# Autodesk Inventor assembly: Housing_Assembly_V4
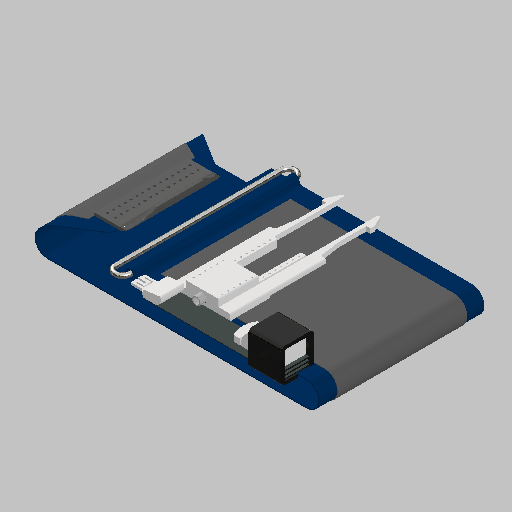
[picture p0: Inventor's stored thumbnail of the model, 512x512]
Saved by Autodesk Inventor 2026.2 (Build 302298000, 298)
## iProperties
Created: 2026-03-15
Part Number: Housing_Assembly_V4
Document SubType Name: Assembly
Designer: vckot
Author: vckot
## Documents named in this file (24)
- C:\Users\vckot\OneDrive\Documents\Vaibhav\capstone\CAD_files\Version_6\Housing_Assembly_V6.iam
- C:\Users\vckot\OneDrive\Documents\Vaibhav\capstone\CAD_files\Version_6\PCB_Housing_01_V4.ipt
- C:\Users\vckot\OneDrive\Documents\Vaibhav\capstone\CAD_files\Version_6\Battery_Small.ipt
- C:\Users\vckot\OneDrive\Documents\Vaibhav\capstone\CAD_files\Version_6\Adafruit_1528_4699_ND.ipt
- C:\Users\vckot\OneDrive\Documents\Vaibhav\capstone\CAD_files\Version_6\Adafruit_1528-4663-ND.ipt
- C:\Users\vckot\OneDrive\Documents\Vaibhav\capstone\CAD_files\Version_6\Adafruit_4662.ipt
- C:\Users\vckot\OneDrive\Documents\Vaibhav\capstone\CAD_files\Version_6\Snap_Switch_Assembly.iam
- C:\Users\vckot\OneDrive\Documents\Vaibhav\capstone\CAD_files\Version_6\PCB_Housing_02_V4.ipt
- C:\Users\vckot\OneDrive\Documents\Vaibhav\capstone\CAD_files\Version_6\PCB_Housing_03_V4.ipt
- C:\Users\vckot\OneDrive\Documents\Vaibhav\capstone\CAD_files\Version_6\PCB_Housing_04_V4.ipt
- C:\Users\vckot\OneDrive\Documents\Vaibhav\capstone\CAD_files\Version_6\TourniquetPCBV1_Updated.iam
- C:\Users\vckot\OneDrive\Documents\Vaibhav\capstone\CAD_files\Version_6\PCB_Housing_05_V4.ipt
- C:\Users\vckot\OneDrive\Documents\Vaibhav\capstone\CAD_files\Version_6\7_Seg_Display_TM1637.ipt
- C:\Users\vckot\OneDrive\Documents\Vaibhav\capstone\CAD_files\Version_6\PCB_Housing_07_V4.ipt
- C:\Users\vckot\OneDrive\Documents\Vaibhav\capstone\CAD_files\Version_6\PCB_Housing_06_V4.ipt
- C:\Users\vckot\OneDrive\Documents\Vaibhav\capstone\CAD_files\Version_6\Tourniquet_Rail_01_V4.ipt
- C:\Users\vckot\OneDrive\Documents\Vaibhav\capstone\CAD_files\Version_6\PCB_Housing_08_V4.ipt
- C:\Users\vckot\OneDrive\Documents\Vaibhav\capstone\CAD_files\Version_6\Tubing_Male_Connector.ipt
- C:\Users\vckot\OneDrive\Documents\Vaibhav\capstone\CAD_files\Version_6\Rail_Tube.ipt
- C:\Users\vckot\OneDrive\Documents\Vaibhav\capstone\CAD_files\Version_6\Cuff_Tube.ipt
- C:\Users\vckot\OneDrive\Documents\Vaibhav\capstone\CAD_files\Version_6\SS-5FL111-3T_Housing_02.ipt
- C:\Users\vckot\OneDrive\Documents\Vaibhav\capstone\CAD_files\Version_6\Inflate_Button.ipt
- C:\Users\vckot\OneDrive\Documents\Vaibhav\capstone\CAD_files\Version_6\Tourniquet_Cuff.ipt
- C:\Users\vckot\OneDrive\Documents\Vaibhav\capstone\CAD_files\Insertion_Slot\Insertion_Slot_V4\Insertion_Slot_V4\Insertion_Slot_V4.ipt
## Components (24 placed, 23 different names)
1. PCB_Housing_01_V4:1 — Flush:1, Flush:2, Flush:3, Mate:1, Flush:4, Flush:5, Mate:2, Angle:1, Mate:11, Mate:13, Mate:14, Flush:7, Flush:8, Mate:17, Mate:25, Flush:14, Flush:15, Flush:16, Mate:34, Mate:37, Flush:17, Mate:47
2. Battery_Small:1 — Mate:1, Flush:4, Flush:5, Flush:6, Mate:3, Mate:15
3. Adafruit_1528_4699_ND:1 — Mate:2, Flush:6, Mate:3, Mate:4, Mate:5
4. Adafruit_1528-4663-ND:1 — Mate:4, Mate:5, Angle:1, Mate:6, Mate:7, Angle:2
5. Adafruit_4662:1 — Mate:6, Mate:7, Angle:2
6. Adafruit_4662:2 — Mate:12, Mate:13
7. Snap_Switch_Assembly:1 [sub-assembly] — Mate:9, Mate:10, Mate:11, Mate:12, Mate:39
8. PCB_Housing_02_V4:1 — Mate:14, Mate:15, Mate:16, Mate:18, Flush:9, Flush:10, Mate:19, Flush:11, Mate:20
9. PCB_Housing_03_V4:1 — Flush:7, Flush:8, Mate:17, Mate:9, Mate:10, Mate:16, Angle:3, Angle:4, Flush:12, Flush:13, Mate:24, Mate:40
10. PCB_Housing_04_V4:1 — Mate:18, Flush:9, Flush:10, Mate:21, Mate:26, Mate:27, Mate:28, Mate:29, Mate:30
11. TourniquetPCBV1_Updated:1 [sub-assembly] — Angle:3, Angle:4, Mate:21, Mate:26, Mate:27
12. PCB_Housing_05_V4:1 — Mate:19, Flush:11, Mate:20
13. 7_Seg_Display_TM1637:1 — Mate:28, Mate:29, Mate:30
14. PCB_Housing_06_V4:1 — Flush:12, Flush:13, Mate:24, Mate:31, Mate:32, Mate:33, Mate:41, Mate:42, Mate:43
15. PCB_Housing_07_V4:1 — Mate:25, Flush:14
16. Tourniquet_Rail_01_V4:1 — Flush:15, Flush:16, Mate:34, Mate:35, Mate:36, Mate:38, Flush:18, Mate:46, Flush:19
17. PCB_Housing_08_V4:1 — Mate:31, Mate:32, Mate:33
18. Tubing_Male_Connector:1 — Mate:35, Mate:36
19. Rail_Tube:1 — Mate:37, Flush:17
20. Cuff_Tube:1 — Mate:38, Flush:18
21. SS-5FL111-3T_Housing_02:1 — Mate:39, Mate:40
22. Inflate_Button:1 — Mate:41, Mate:42, Mate:43
23. Tourniquet_Cuff:1 — Mate:44, Angle:5, Mate:45, Mate:46, Mate:47, Flush:19, Flush:20
24. Insertion_Slot_V4:1 — Mate:44, Angle:5, Mate:45, Flush:20
## Relationships (69: Mate 44, Flush 20, Angle 5)
- Flush:1: PCB_Housing_01_V4:1
- Flush:2: PCB_Housing_01_V4:1
- Flush:3: PCB_Housing_01_V4:1
- Mate:1: PCB_Housing_01_V4:1 ↔ Battery_Small:1
- Flush:4 (2.5 mm): PCB_Housing_01_V4:1 ↔ Battery_Small:1
- Flush:5 (2.5 mm): PCB_Housing_01_V4:1 ↔ Battery_Small:1
- Mate:2 (1 mm): PCB_Housing_01_V4:1 ↔ Adafruit_1528_4699_ND:1
- Flush:6 (4 mm): Battery_Small:1 ↔ Adafruit_1528_4699_ND:1
- Mate:3 (18 mm): Battery_Small:1 ↔ Adafruit_1528_4699_ND:1
- Mate:4: Adafruit_1528_4699_ND:1 ↔ Adafruit_1528-4663-ND:1
- Mate:5 (1 mm): Adafruit_1528_4699_ND:1 ↔ Adafruit_1528-4663-ND:1
- Angle:1 (180 deg): PCB_Housing_01_V4:1 ↔ Adafruit_1528-4663-ND:1
- Mate:6: Adafruit_1528-4663-ND:1 ↔ Adafruit_4662:1
- Mate:7 (5 mm): Adafruit_1528-4663-ND:1 ↔ Adafruit_4662:1
- Angle:2 (45 deg): Adafruit_1528-4663-ND:1 ↔ Adafruit_4662:1
- Mate:9: Snap_Switch_Assembly:1 ↔ PCB_Housing_03_V4:1
- Mate:10: Snap_Switch_Assembly:1 ↔ PCB_Housing_03_V4:1
- Mate:11: PCB_Housing_01_V4:1 ↔ Snap_Switch_Assembly:1
- Mate:12: Adafruit_4662:2 ↔ Snap_Switch_Assembly:1
- Mate:13: PCB_Housing_01_V4:1 ↔ Adafruit_4662:2
- Mate:14: PCB_Housing_01_V4:1 ↔ PCB_Housing_02_V4:1
- Mate:15: Battery_Small:1 ↔ PCB_Housing_02_V4:1
- Mate:16 (2 mm): PCB_Housing_02_V4:1 ↔ PCB_Housing_03_V4:1
- Flush:7: PCB_Housing_01_V4:1 ↔ PCB_Housing_03_V4:1
- Flush:8: PCB_Housing_01_V4:1 ↔ PCB_Housing_03_V4:1
- Mate:17: PCB_Housing_01_V4:1 ↔ PCB_Housing_03_V4:1
- Mate:18: PCB_Housing_02_V4:1 ↔ PCB_Housing_04_V4:1
- Flush:9: PCB_Housing_02_V4:1 ↔ PCB_Housing_04_V4:1
- Flush:10: PCB_Housing_02_V4:1 ↔ PCB_Housing_04_V4:1
- Angle:3 (0 deg): PCB_Housing_03_V4:1 ↔ TourniquetPCBV1_Updated:1
- Angle:4 (0 deg): PCB_Housing_03_V4:1 ↔ TourniquetPCBV1_Updated:1
- Mate:19: PCB_Housing_02_V4:1 ↔ PCB_Housing_05_V4:1
- Flush:11: PCB_Housing_02_V4:1 ↔ PCB_Housing_05_V4:1
- Mate:20 (2.5 mm): PCB_Housing_02_V4:1 ↔ PCB_Housing_05_V4:1
- Mate:21: PCB_Housing_04_V4:1 ↔ TourniquetPCBV1_Updated:1
- Flush:12: PCB_Housing_03_V4:1 ↔ PCB_Housing_06_V4:1
- Flush:13: PCB_Housing_03_V4:1 ↔ PCB_Housing_06_V4:1
- Mate:24: PCB_Housing_03_V4:1 ↔ PCB_Housing_06_V4:1
- Mate:25: PCB_Housing_01_V4:1 ↔ PCB_Housing_07_V4:1
- Flush:14: PCB_Housing_01_V4:1 ↔ PCB_Housing_07_V4:1
- Flush:15: PCB_Housing_01_V4:1 ↔ Tourniquet_Rail_01_V4:1
- Flush:16: PCB_Housing_01_V4:1 ↔ Tourniquet_Rail_01_V4:1
- Mate:26: PCB_Housing_04_V4:1 ↔ TourniquetPCBV1_Updated:1
- Mate:27: PCB_Housing_04_V4:1 ↔ TourniquetPCBV1_Updated:1
- Mate:28 (2 mm): PCB_Housing_04_V4:1 ↔ 7_Seg_Display_TM1637:1
- Mate:29: PCB_Housing_04_V4:1 ↔ 7_Seg_Display_TM1637:1
- Mate:30: PCB_Housing_04_V4:1 ↔ 7_Seg_Display_TM1637:1
- Mate:31: PCB_Housing_06_V4:1 ↔ PCB_Housing_08_V4:1
- Mate:32: PCB_Housing_06_V4:1 ↔ PCB_Housing_08_V4:1
- Mate:33: PCB_Housing_06_V4:1 ↔ PCB_Housing_08_V4:1
- Mate:34: PCB_Housing_01_V4:1 ↔ Tourniquet_Rail_01_V4:1
- Mate:35: Tourniquet_Rail_01_V4:1 ↔ Tubing_Male_Connector:1
- Mate:36 (12 mm): Tourniquet_Rail_01_V4:1 ↔ Tubing_Male_Connector:1
- Mate:37: PCB_Housing_01_V4:1 ↔ Rail_Tube:1
- Flush:17 (-2 mm): PCB_Housing_01_V4:1 ↔ Rail_Tube:1
- Mate:38: Tourniquet_Rail_01_V4:1 ↔ Cuff_Tube:1
- Flush:18 (-5 mm): Tourniquet_Rail_01_V4:1 ↔ Cuff_Tube:1
- Mate:39: Snap_Switch_Assembly:1 ↔ SS-5FL111-3T_Housing_02:1
- Mate:40: PCB_Housing_03_V4:1 ↔ SS-5FL111-3T_Housing_02:1
- Mate:41: PCB_Housing_06_V4:1 ↔ Inflate_Button:1
- Mate:42 (3.5 mm): PCB_Housing_06_V4:1 ↔ Inflate_Button:1
- Mate:43 (3.5 mm): PCB_Housing_06_V4:1 ↔ Inflate_Button:1
- Mate:44: Tourniquet_Cuff:1 ↔ Insertion_Slot_V4:1
- Angle:5 (180 deg): Tourniquet_Cuff:1 ↔ Insertion_Slot_V4:1
- Mate:45: Tourniquet_Cuff:1 ↔ Insertion_Slot_V4:1
- Mate:46: Tourniquet_Rail_01_V4:1 ↔ Tourniquet_Cuff:1
- Mate:47: PCB_Housing_01_V4:1 ↔ Tourniquet_Cuff:1
- Flush:19 (10 mm): Tourniquet_Rail_01_V4:1 ↔ Tourniquet_Cuff:1
- Flush:20 (30 mm): Tourniquet_Cuff:1 ↔ Insertion_Slot_V4:1
